# Autodesk Inventor assembly: FinalBlueSail-ver1-1111-2021
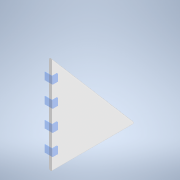
[picture p0: Inventor's stored thumbnail of the model, 180x180]
Saved by Autodesk Inventor 2021 (Build 250183000, 183)
## iProperties
Created: 2021-03-03
Part Number: FinalBlueSail-ver1-1111-2021
Document SubType Name: Assembly
Designer: CMurray
Author: CMurray
## Documents named in this file (3)
- F:\PHRC CADD 2021\2021 Game Design Challenge\Sail\Assemblies\FinalBlueSail-ver1-1111-2021.iam
- F:\PHRC CADD 2021\2021 Game Design Challenge\Sail\Parts\RedSail-ver1-1111-2021.ipt
- F:\PHRC CADD 2021\2021 Game Design Challenge\Sail\Parts\BlueLights-ver-1-1111-2021.ipt
## Components (2 placed, 2 different names)
1. RedSail-ver1-1111-2021:1 — Mate:3, Mate:4, Flush:3
2. BlueLights-ver-1-1111-2021:1 — Mate:3, Mate:4, Flush:3
## Relationships (3: Mate 2, Flush 1)
- Mate:3: RedSail-ver1-1111-2021:1 ↔ BlueLights-ver-1-1111-2021:1
- Mate:4: RedSail-ver1-1111-2021:1 ↔ BlueLights-ver-1-1111-2021:1
- Flush:3 (292.1 mm): RedSail-ver1-1111-2021:1 ↔ BlueLights-ver-1-1111-2021:1
